# Autodesk Inventor assembly: mount assem
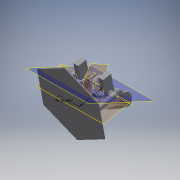
[picture p0: Inventor's stored thumbnail of the model, 180x180]
Saved by Autodesk Inventor 2019.3 (Build 233278000, 278)
## iProperties
Created: 2018-10-05
Part Number: mount assem
Document SubType Name: Assembly
Designer: HIVE
Author: HIVE
## Documents named in this file (5)
- D:\hive\projects\pocketpelvis\models\mounts\V2\femur\old stuff\mount assem.iam
- D:\hive\projects\pocketpelvis\models\mounts\V2\femur\old stuff\3945K300_HIGH-PULL RARE EARTH MAGNETIC BALL.ipt
- D:\hive\projects\pocketpelvis\models\mounts\V2\femur\old stuff\mounter.ipt
- D:\hive\projects\pocketpelvis\models\mounts\V2\Imported Components\pelvis_scaled1point6\pelvis_scaled1point6.ipt
- D:\hive\projects\pocketpelvis\models\mounts\V2\femur\clip and shaft assem.iam
## Components (5 placed, 4 different names)
1. pelvis_scaled1point6:2
2. 3945K300_HIGH-PULL RARE EARTH MAGNETIC BALL:1 — Mate:3
3. 3945K300_HIGH-PULL RARE EARTH MAGNETIC BALL:2 — Mate:4
4. mounter:1 — Mate:8, Mate:10, Mate:11, Angle:2
5. clip and shaft assem:1 [sub-assembly] — Mate:11, Mate:12, Angle:2
## Relationships (10: Mate 8, Angle 2)
- Mate:3: 3945K300_HIGH-PULL RARE EARTH MAGNETIC BALL:1
- Mate:4: 3945K300_HIGH-PULL RARE EARTH MAGNETIC BALL:2
- Mate:5
- Mate:6
- Mate:8: mounter:1
- Mate:10: mounter:1
- Angle:1 (-155 deg)
- Mate:11: mounter:1 ↔ clip and shaft assem:1
- Mate:12: clip and shaft assem:1
- Angle:2 (-90 deg): mounter:1 ↔ clip and shaft assem:1
